# Autodesk Inventor assembly: Nanoscopy-on-a-cheap_v4_nanomax
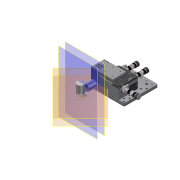
[picture p0: Inventor's stored thumbnail of the model, 180x180]
Saved by Autodesk Inventor 2019 (Build 230136000, 136)
## iProperties
Created: 2019-06-11
Part Number: Nanoscopy-on-a-cheap_v4_nanomax
Document SubType Name: Assembly
Designer: diederichbenedict
Author: diederichbenedict
## Documents named in this file (7)
- C:\Users\diederichbenedict\Dropbox\Dokumente\Promotion\PROJECTS\STORMoChip\INVENTOR\Nanoscopy-on-a-cheap\Nanoscopy-on-a-cheap_v4_nanomax.iam
- C:\Users\diederichbenedict\Dropbox\Dokumente\Promotion\PROJECTS\STORMoChip\INVENTOR\Nanoscopy-on-a-cheap\MAX313D_M-Step.ipt
- C:\Users\diederichbenedict\Dropbox\Dokumente\Promotion\PROJECTS\STORMoChip\INVENTOR\Nanoscopy-on-a-cheap\MB1515_M-Step.ipt
- C:\Users\diederichbenedict\Dropbox\Dokumente\Promotion\PROJECTS\STORMoChip\INVENTOR\Nanoscopy-on-a-cheap\00_Microscope_Objective.ipt
- C:\Users\diederichbenedict\Dropbox\Dokumente\Promotion\PROJECTS\STORMoChip\INVENTOR\Nanoscopy-on-a-cheap\00_LASER_640nm.ipt
- C:\Users\diederichbenedict\Dropbox\Dokumente\Promotion\PROJECTS\STORMoChip\INVENTOR\Nanoscopy-on-a-cheap\02_Nanoscopy_Chip.ipt
- C:\Users\diederichbenedict\Dropbox\Dokumente\Promotion\PROJECTS\STORMoChip\INVENTOR\Nanoscopy-on-a-cheap\04_Bridge_Laser_Nanomax.ipt
## Components (7 placed, 6 different names)
1. MAX313D_M-Step:1 — Insert:1, Angle:1, Mate:3, Flush:1, Flush:2, Flush:3
2. MB1515_M-Step:1 — Insert:1, Angle:1, Mate:2, Angle:2
3. 00_Microscope_Objective:1 — Insert:3
4. 00_LASER_640nm:1 — Mate:2, Flush:1, Insert:2, Mate:3
5. 00_Microscope_Objective:2 — Insert:2
6. 02_Nanoscopy_Chip:1 — Insert:3, Angle:2
7. 04_Bridge_Laser_Nanomax:1 — Flush:2, Flush:3
## Relationships (10: Insert 3, Flush 3, Angle 2, Mate 2)
- Insert:1: MAX313D_M-Step:1 ↔ MB1515_M-Step:1
- Angle:1 (180 deg): MAX313D_M-Step:1 ↔ MB1515_M-Step:1
- Mate:2 (2 mm): MB1515_M-Step:1 ↔ 00_LASER_640nm:1
- Flush:1: MAX313D_M-Step:1 ↔ 00_LASER_640nm:1
- Insert:2 (15 mm): 00_LASER_640nm:1 ↔ 00_Microscope_Objective:2
- Insert:3 (3 mm): 00_Microscope_Objective:1 ↔ 02_Nanoscopy_Chip:1
- Angle:2 (90 deg): MB1515_M-Step:1 ↔ 02_Nanoscopy_Chip:1
- Mate:3 (5 mm): MAX313D_M-Step:1 ↔ 00_LASER_640nm:1
- Flush:2: MAX313D_M-Step:1 ↔ 04_Bridge_Laser_Nanomax:1
- Flush:3: MAX313D_M-Step:1 ↔ 04_Bridge_Laser_Nanomax:1
